# Autodesk Inventor assembly: Intake Assembly
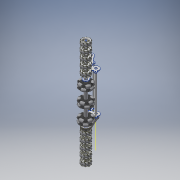
[picture p0: Inventor's stored thumbnail of the model, 180x180]
Saved by Autodesk Inventor 2019.4 (Build 234330000, 330)
## iProperties
Created: 2020-01-28
Part Number: Intake Assembly
Document SubType Name: Assembly
Designer: admin
Mass: 1824.68 g
Surface Area: 5963.11 cm^2
Volume: 979.583 cm^3
Density: 1.86271 g/cm^3
Author: admin
## Documents named in this file (14)
- C:\Users\admin\Desktop\FRC 2020 Engineering\GitHub\7738-2020\Robot V2\Intake V2\Intake Assembly.iam
- C:\Users\admin\Desktop\FRC 2020 Engineering\GitHub\7738-2020\Robot V2\Intake V2\Intake Arm.ipt
- C:\Users\admin\Desktop\FRC 2020 Engineering\GitHub\7738-2020\Robot V2\Intake V2\Omni Wheel\3_25_Omni-Directional_Wheel_217-4775.iam
- C:\Users\admin\Desktop\FRC 2020 Engineering\GitHub\7738-2020\Robot V2\Turret\775\775pro_775pro_Connect_and_GT2_Pulley_217-6347 (1).iam
- C:\Users\admin\Desktop\FRC 2020 Engineering\GitHub\7738-2020\Robot V2\Intake V2\Intake Assembly\Design Accelerator\Synchronous Belts Transmission1.iam
- C:\Users\admin\Desktop\FRC 2020 Engineering\GitHub\7738-2020\Robot V2\Intake System\MF148ZZ.ipt
- C:\Users\admin\Desktop\FRC 2020 Engineering\GitHub\7738-2020\Robot V2\Turret\F6800.ipt
- C:\Users\admin\Desktop\FRC 2020 Engineering\GitHub\7738-2020\Robot V2\Intake V2\Mecanum Rad 58x27 Rechts 23 rollen v6.iam
- C:\Users\admin\Desktop\FRC 2020 Engineering\GitHub\7738-2020\Robot V2\Intake V2\Saftey Axle.ipt
- C:\Users\admin\Desktop\FRC 2020 Engineering\GitHub\7738-2020\Robot V2\Intake V2\Intake Plate Spacer.ipt
- C:\Users\admin\Desktop\FRC 2020 Engineering\GitHub\7738-2020\Robot V2\Intake V2\Intake Axle.ipt
- C:\Users\admin\Desktop\FRC 2020 Engineering\GitHub\7738-2020\Robot V2\Intake V2\Mec Wheel Spacer.ipt
- C:\Users\admin\Desktop\FRC 2020 Engineering\GitHub\7738-2020\Robot V2\Intake V2\Omni Wheel Spacer.ipt
- C:\Users\admin\Desktop\FRC 2020 Engineering\GitHub\7738-2020\Robot V2\Intake V2\Omni Wheel Spacer 2.ipt
## Components (39 placed, 13 different names)
1. Intake Arm:1 — Mate:1, Mate:2, Mate:3, Mate:4, Mate:5, Mate:6, Mate:7, Mate:9, Mate:10, Mate:11, Mate:13, Mate:15, Mate:18, Mate:23, Mate:60, Mate:61, Mate:65, Mate:66, Mate:67, Mate:68, Mate:84
2. Intake Arm:2 — Mate:1, Mate:2, Mate:3, Mate:8, Mate:16, Mate:17, Mate:21, Mate:22, Mate:42, Mate:55, Mate:56, Mate:57, Mate:58, Mate:59, Mate:62, Mate:77, Mate:78, Mate:79, Mate:80, Mate:82
3. 3_25_Omni-Directional_Wheel_217-4775:1 [sub-assembly] — Mate:4, Mate:47, Mate:86, Mate:88, Mate:89
4. 3_25_Omni-Directional_Wheel_217-4775:2 [sub-assembly] — Mate:5, Mate:90
5. 3_25_Omni-Directional_Wheel_217-4775:3 [sub-assembly] — Mate:6, Mate:52, Mate:85, Mate:87
6. 775pro_775pro_Connect_and_GT2_Pulley_217-6347 (1):1 [sub-assembly] — Mate:9, Mate:10, Mate:23
7. Synchronous Belts Transmission:1 [sub-assembly] — Mate:30
8. MF148ZZ:2 — Mate:11, Mate:13, Mate:53, Mate:54
9. F6800:1 — Mate:15, Mate:18
10. F6800:2 — Mate:16, Mate:17
11. MF148ZZ:4 — Mate:21, Mate:22
12. Mecanum Rad 58x27 Rechts 23 rollen v6:4 [sub-assembly] — Mate:29, Mate:31, Mate:43, Mate:44, Mate:70
13. Mecanum Rad 58x27 Rechts 23 rollen v6:5 [sub-assembly] — Mate:33, Mate:46
14. Mecanum Rad 58x27 Rechts 23 rollen v6:6 [sub-assembly] — Mate:31, Mate:32, Mate:44, Mate:45, Mate:71
15. Mecanum Rad 58x27 Rechts 23 rollen v6:7 [sub-assembly] — Mate:32, Mate:33, Mate:45, Mate:46, Mate:72
16. Mecanum Rad 58x27 Rechts 23 rollen v6:8 [sub-assembly] — Mate:29, Mate:30, Mate:43, Mate:47, Mate:69
17. Mecanum Rad 58x27 Rechts 23 rollen v6:9 [sub-assembly] — Mate:48, Mate:49, Mate:74
18. Mecanum Rad 58x27 Rechts 23 rollen v6:10 [sub-assembly] — Mate:51
19. Mecanum Rad 58x27 Rechts 23 rollen v6:11 [sub-assembly] — Mate:49, Mate:50, Mate:75
20. Mecanum Rad 58x27 Rechts 23 rollen v6:12 [sub-assembly] — Mate:50, Mate:51, Mate:76
21. Mecanum Rad 58x27 Rechts 23 rollen v6:13 [sub-assembly] — Mate:42, Mate:48, Mate:52, Mate:73
22. Saftey Axle:1 — Mate:53, Mate:54
23. Intake Plate Spacer:1 — Mate:55, Mate:57
24. Intake Plate Spacer:2 — Mate:56, Mate:58
25. F6800:3 — Mate:59, Mate:62, Mate:63, Mate:64, Mate:81
26. F6800:4 — Mate:60, Mate:61, Mate:83
27. Intake Axle:1 — Mate:63, Mate:64
28. Mec Wheel Spacer:1 — Mate:65, Mate:71
29. Mec Wheel Spacer:2 — Mate:66, Mate:70
30. Mec Wheel Spacer:3 — Mate:67, Mate:72
31. Mec Wheel Spacer:4 — Mate:68, Mate:69
32. Mec Wheel Spacer:5 — Mate:76, Mate:80
33. Mec Wheel Spacer:6 — Mate:75, Mate:79
34. Mec Wheel Spacer:7 — Mate:74, Mate:78
35. Mec Wheel Spacer:8 — Mate:73, Mate:77
36. Omni Wheel Spacer:1 — Mate:81, Mate:82, Mate:85
37. Omni Wheel Spacer:2 — Mate:83, Mate:84, Mate:86
38. Omni Wheel Spacer 2:1 — Mate:87, Mate:90
39. Omni Wheel Spacer 2:2 — Mate:88, Mate:89
## Relationships (77: Mate 77)
- Mate:1: Intake Arm:1 ↔ Intake Arm:2
- Mate:2: Intake Arm:1 ↔ Intake Arm:2
- Mate:3 (248.6 mm): Intake Arm:1 ↔ Intake Arm:2
- Mate:4: Intake Arm:1 ↔ 3_25_Omni-Directional_Wheel_217-4775:1
- Mate:5: Intake Arm:1 ↔ 3_25_Omni-Directional_Wheel_217-4775:2
- Mate:6: Intake Arm:1 ↔ 3_25_Omni-Directional_Wheel_217-4775:3
- Mate:7: Intake Arm:1
- Mate:8 (119.3 mm): Intake Arm:2
- Mate:9: Intake Arm:1 ↔ 775pro_775pro_Connect_and_GT2_Pulley_217-6347 (1):1
- Mate:10: Intake Arm:1 ↔ 775pro_775pro_Connect_and_GT2_Pulley_217-6347 (1):1
- Mate:11: Intake Arm:1 ↔ MF148ZZ:2
- Mate:13 (0.2 mm): Intake Arm:1 ↔ MF148ZZ:2
- Mate:15: Intake Arm:1 ↔ F6800:1
- Mate:16: Intake Arm:2 ↔ F6800:2
- Mate:17 (0.2 mm): Intake Arm:2 ↔ F6800:2
- Mate:18 (0.2 mm): Intake Arm:1 ↔ F6800:1
- Mate:21: Intake Arm:2 ↔ MF148ZZ:4
- Mate:22 (0.2 mm): Intake Arm:2 ↔ MF148ZZ:4
- Mate:23: Intake Arm:1 ↔ 775pro_775pro_Connect_and_GT2_Pulley_217-6347 (1):1
- Mate:29 (20 mm): Mecanum Rad 58x27 Rechts 23 rollen v6:4 ↔ Mecanum Rad 58x27 Rechts 23 rollen v6:8
- Mate:30 (5 mm): Synchronous Belts Transmission:1 ↔ Mecanum Rad 58x27 Rechts 23 rollen v6:8
- Mate:31 (20 mm): Mecanum Rad 58x27 Rechts 23 rollen v6:4 ↔ Mecanum Rad 58x27 Rechts 23 rollen v6:6
- Mate:32 (20 mm): Mecanum Rad 58x27 Rechts 23 rollen v6:6 ↔ Mecanum Rad 58x27 Rechts 23 rollen v6:7
- Mate:33 (20 mm): Mecanum Rad 58x27 Rechts 23 rollen v6:5 ↔ Mecanum Rad 58x27 Rechts 23 rollen v6:7
- [Mate] (20 mm): Mecanum Rad 58x27 Rechts 23 rollen v6:9 ↔ Mecanum Rad 58x27 Rechts 23 rollen v6:13
- [Mate] (20 mm): Mecanum Rad 58x27 Rechts 23 rollen v6:9 ↔ Mecanum Rad 58x27 Rechts 23 rollen v6:11
- [Mate] (20 mm): Mecanum Rad 58x27 Rechts 23 rollen v6:11 ↔ Mecanum Rad 58x27 Rechts 23 rollen v6:12
- [Mate] (20 mm): Mecanum Rad 58x27 Rechts 23 rollen v6:10 ↔ Mecanum Rad 58x27 Rechts 23 rollen v6:12
- Mate:42 (22.5 mm): Intake Arm:2 ↔ Mecanum Rad 58x27 Rechts 23 rollen v6:13
- Mate:43: Mecanum Rad 58x27 Rechts 23 rollen v6:4 ↔ Mecanum Rad 58x27 Rechts 23 rollen v6:8
- Mate:44: Mecanum Rad 58x27 Rechts 23 rollen v6:4 ↔ Mecanum Rad 58x27 Rechts 23 rollen v6:6
- Mate:45: Mecanum Rad 58x27 Rechts 23 rollen v6:6 ↔ Mecanum Rad 58x27 Rechts 23 rollen v6:7
- Mate:46: Mecanum Rad 58x27 Rechts 23 rollen v6:5 ↔ Mecanum Rad 58x27 Rechts 23 rollen v6:7
- Mate:47: 3_25_Omni-Directional_Wheel_217-4775:1 ↔ Mecanum Rad 58x27 Rechts 23 rollen v6:8
- Mate:48: Mecanum Rad 58x27 Rechts 23 rollen v6:9 ↔ Mecanum Rad 58x27 Rechts 23 rollen v6:13
- Mate:49: Mecanum Rad 58x27 Rechts 23 rollen v6:9 ↔ Mecanum Rad 58x27 Rechts 23 rollen v6:11
- Mate:50: Mecanum Rad 58x27 Rechts 23 rollen v6:11 ↔ Mecanum Rad 58x27 Rechts 23 rollen v6:12
- Mate:51: Mecanum Rad 58x27 Rechts 23 rollen v6:10 ↔ Mecanum Rad 58x27 Rechts 23 rollen v6:12
- Mate:52: 3_25_Omni-Directional_Wheel_217-4775:3 ↔ Mecanum Rad 58x27 Rechts 23 rollen v6:13
- Mate:53: MF148ZZ:2 ↔ Saftey Axle:1
- Mate:54: MF148ZZ:2 ↔ Saftey Axle:1
- Mate:55: Intake Arm:2 ↔ Intake Plate Spacer:1
- Mate:56: Intake Arm:2 ↔ Intake Plate Spacer:2
- Mate:57: Intake Arm:2 ↔ Intake Plate Spacer:1
- Mate:58: Intake Arm:2 ↔ Intake Plate Spacer:2
- Mate:59: Intake Arm:2 ↔ F6800:3
- Mate:60: Intake Arm:1 ↔ F6800:4
- Mate:61 (0.2 mm): Intake Arm:1 ↔ F6800:4
- Mate:62 (0.2 mm): Intake Arm:2 ↔ F6800:3
- Mate:63: F6800:3 ↔ Intake Axle:1
- Mate:64: F6800:3 ↔ Intake Axle:1
- Mate:65: Intake Arm:1 ↔ Mec Wheel Spacer:1
- Mate:66: Intake Arm:1 ↔ Mec Wheel Spacer:2
- Mate:67: Intake Arm:1 ↔ Mec Wheel Spacer:3
- Mate:68: Intake Arm:1 ↔ Mec Wheel Spacer:4
- Mate:69 (0.2 mm): Mecanum Rad 58x27 Rechts 23 rollen v6:8 ↔ Mec Wheel Spacer:4
- Mate:70 (0.2 mm): Mecanum Rad 58x27 Rechts 23 rollen v6:4 ↔ Mec Wheel Spacer:2
- Mate:71 (0.2 mm): Mecanum Rad 58x27 Rechts 23 rollen v6:6 ↔ Mec Wheel Spacer:1
- Mate:72 (0.2 mm): Mecanum Rad 58x27 Rechts 23 rollen v6:7 ↔ Mec Wheel Spacer:3
- Mate:73 (0.2 mm): Mecanum Rad 58x27 Rechts 23 rollen v6:13 ↔ Mec Wheel Spacer:8
- Mate:74 (0.2 mm): Mecanum Rad 58x27 Rechts 23 rollen v6:9 ↔ Mec Wheel Spacer:7
- Mate:75 (0.2 mm): Mecanum Rad 58x27 Rechts 23 rollen v6:11 ↔ Mec Wheel Spacer:6
- Mate:76 (0.2 mm): Mecanum Rad 58x27 Rechts 23 rollen v6:12 ↔ Mec Wheel Spacer:5
- Mate:77: Intake Arm:2 ↔ Mec Wheel Spacer:8
- Mate:78: Intake Arm:2 ↔ Mec Wheel Spacer:7
- Mate:79: Intake Arm:2 ↔ Mec Wheel Spacer:6
- Mate:80: Intake Arm:2 ↔ Mec Wheel Spacer:5
- Mate:81: F6800:3 ↔ Omni Wheel Spacer:1
- Mate:82: Intake Arm:2 ↔ Omni Wheel Spacer:1
- Mate:83: F6800:4 ↔ Omni Wheel Spacer:2
- Mate:84: Intake Arm:1 ↔ Omni Wheel Spacer:2
- Mate:85 (0.4 mm): 3_25_Omni-Directional_Wheel_217-4775:3 ↔ Omni Wheel Spacer:1
- Mate:86 (0.4 mm): 3_25_Omni-Directional_Wheel_217-4775:1 ↔ Omni Wheel Spacer:2
- Mate:87: 3_25_Omni-Directional_Wheel_217-4775:3 ↔ Omni Wheel Spacer 2:1
- Mate:88: 3_25_Omni-Directional_Wheel_217-4775:1 ↔ Omni Wheel Spacer 2:2
- Mate:89: 3_25_Omni-Directional_Wheel_217-4775:1 ↔ Omni Wheel Spacer 2:2
- Mate:90: 3_25_Omni-Directional_Wheel_217-4775:2 ↔ Omni Wheel Spacer 2:1
